# Autodesk Inventor assembly: prototype7
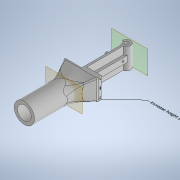
[picture p0: Inventor's stored thumbnail of the model, 180x180]
Saved by Autodesk Inventor 2022 (Build 260153000, 153)
## iProperties
Created: 2022-06-15
Part Number: prototype7
Document SubType Name: Assembly
Designer: tecware
Author: tecware
## Documents named in this file (4)
- C:\Users\tecware\Documents\git\calibrationKit\calibrationKit_v2\wand\prototype\prototype_10.iam
- C:\Users\tecware\Documents\git\calibrationKit\calibrationKit_v2\wand\prototype\prototype_10_1.ipt
- C:\Users\tecware\Documents\git\calibrationKit\calibrationKit_v2\wand\prototype\prototype_10_2.ipt
- C:\Users\tecware\Documents\git\calibrationKit\calibrationKit_v2\wand\prototype\prototype_10_3.ipt
## Components (3 placed, 3 different names)
1. prototype_10_1:1 — Flush:1, Flush:2, Mate:1
2. prototype_10_2:1 — Flush:1, Flush:2, Mate:1
3. prototype_10_3:1
## Relationships (3: Flush 2, Mate 1)
- Flush:1: prototype_10_1:1 ↔ prototype_10_2:1
- Flush:2: prototype_10_1:1 ↔ prototype_10_2:1
- Mate:1 (0.2 mm): prototype_10_1:1 ↔ prototype_10_2:1
